# Autodesk Inventor assembly: SquareSupport
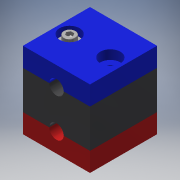
[picture p0: Inventor's stored thumbnail of the model, 180x180]
Saved by Autodesk Inventor 2016 SP1 (Build 200210100, 210)
## iProperties
Created: 2015-12-11
Part Number: SquareSupport
Document SubType Name: Assembly
Designer: steele
Author: steele
## Documents named in this file (5)
- C:\snobotics\CAD-Development\robSteele\HouseProjects\Garage\SquareSupport.iam
- C:\snobotics\CAD-Development\robSteele\HouseProjects\Garage\BottomOfSquareSupport.ipt
- C:\snobotics\CAD-Development\robSteele\HouseProjects\Garage\MiddleOfSquareSupport.ipt
- C:\snobotics\CAD-Development\robSteele\HouseProjects\Garage\TopOfSquareSupport.ipt
- C:\snobotics\CAD-Development\robSteele\HouseProjects\Garage\SquareSupport\Design Accelerator\Bolted Connection2.iam
## Components (4 placed, 4 different names)
1. BottomOfSquareSupport:1 — Mate:1, Flush:1, Flush:2
2. MiddleOfSquareSupport:1 — Mate:1, Flush:1, Flush:2, Mate:5, Flush:3, Flush:4
3. TopOfSquareSupport:1 — Mate:5, Flush:3, Flush:4, Mate:6, Mate:7
4. Bolted Connection:1 [sub-assembly] — Mate:6, Mate:7
## Relationships (8: Mate 4, Flush 4)
- Mate:1: BottomOfSquareSupport:1 ↔ MiddleOfSquareSupport:1
- Flush:1: BottomOfSquareSupport:1 ↔ MiddleOfSquareSupport:1
- Flush:2: BottomOfSquareSupport:1 ↔ MiddleOfSquareSupport:1
- Mate:5: MiddleOfSquareSupport:1 ↔ TopOfSquareSupport:1
- Flush:3: MiddleOfSquareSupport:1 ↔ TopOfSquareSupport:1
- Flush:4: MiddleOfSquareSupport:1 ↔ TopOfSquareSupport:1
- Mate:6: TopOfSquareSupport:1 ↔ Bolted Connection:1
- Mate:7: TopOfSquareSupport:1 ↔ Bolted Connection:1
## Named parameters: bottomHoleDiam = 9.525 mm, width = 38.1 mm, heightOfBottomHole = 11.1125 mm, deltaBottomToTop = 25.4 mm, heightOfTopHole = 11.1125 mm, topHoleDiam = 9.525 mm, edgeToBoltHole = 7.14375 mm, height = 47.625 mm
